# Autodesk Inventor assembly: stand_arbeit
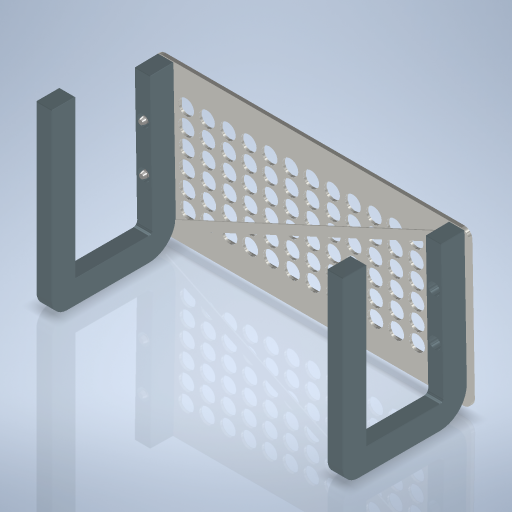
[picture p0: Inventor's stored thumbnail of the model, 512x512]
Saved by Autodesk Inventor 2024 (Build 280153000, 153)
## iProperties
Created: 2024-04-23
Part Number: stand_arbeit
Document SubType Name: Assembly
Designer: ffogue
Mass: 10946.1 g
Surface Area: 2435.39 cm^2
Volume: 819.899 cm^3
Density: 13.3505 g/cm^3
Author: ffogue
## Documents named in this file (10)
- C:\Users\ffogue\OneDrive - MuM - OM\Dokumente\Inventor\Learning\stand_arbeit.iam
- C:\Users\ffogue\OneDrive - MuM - OM\Dokumente\Inventor\Learning\laptopstand.ipt
- C:\Users\ffogue\OneDrive - MuM - OM\Dokumente\Inventor\Learning\plate.ipt
- C:\Users\ffogue\OneDrive - MuM - OM\Dokumente\Inventor\Content Center Files\R2024\de-DE\ANSI B18.6.4(281)\ANSI B18.6.4 - 5_16-12 - 1,5(22) BT.ipt
- C:\Users\ffogue\OneDrive - MuM - OM\Dokumente\Inventor\Learning\stand_arbeit\AIP\FEA\eog9zihvk.fins
- C:\Users\ffogue\OneDrive - MuM - OM\Dokumente\Inventor\Learning\stand_arbeit\AIP\FEA\eog9zihvk.fsat
- C:\Users\ffogue\OneDrive - MuM - OM\Dokumente\Inventor\Learning\stand_arbeit\AIP\FEA\eog9zihvk.ftes
- C:\Users\ffogue\OneDrive - MuM - OM\Dokumente\Inventor\Learning\stand_arbeit\AIP\FEA\eog9zihvk.fwiz
- C:\Users\ffogue\OneDrive - MuM - OM\Dokumente\Inventor\Learning\stand_arbeit\AIP\FEA\eog9zihy8.fmsh
- C:\Users\ffogue\OneDrive - MuM - OM\Dokumente\Inventor\Learning\stand_arbeit\AIP\FEA\eog9zihy9.fres
## Components (5 placed, 3 different names)
1. laptopstand:1 — Einfügen:1
2. plate:2 — Einfügen:1, Einfügen:2, Einfügen:3, Einfügen:4
3. laptopstand:2 — Einfügen:2
4. Sechskantblechschraube mit Schlitz, Vertiefung und Flansch - Form BT - Zoll 5/16-12 - 1,5:1 — Einfügen:3
5. Sechskantblechschraube mit Schlitz, Vertiefung und Flansch - Form BT - Zoll 5/16-12 - 1,5:2 — Einfügen:4
## Relationships (4: Insert 4)
- Einfügen:1 [Insert]: laptopstand:1 ↔ plate:2
- Einfügen:2 [Insert]: plate:2 ↔ laptopstand:2
- Einfügen:3 [Insert] (-33.7 mm): plate:2 ↔ Sechskantblechschraube mit Schlitz, Vertiefung und Flansch - Form BT - Zoll 5/16-12 - 1,5:1
- Einfügen:4 [Insert] (-33.5 mm): plate:2 ↔ Sechskantblechschraube mit Schlitz, Vertiefung und Flansch - Form BT - Zoll 5/16-12 - 1,5:2
